# Autodesk Inventor assembly: 0304_練習
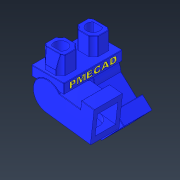
[picture p0: Inventor's stored thumbnail of the model, 180x180]
Saved by Autodesk Inventor 2022 (Build 260153000, 153)
## iProperties
Created: 2022-03-04
Part Number: 0304_練習
Document SubType Name: Assembly
Designer: user
Author: user
## Documents named in this file (4)
- D:\pomelo\大一\下學期\機械設計製圖\PME1017_110033226\0304_練習.iam
- D:\pomelo\大一\下學期\機械設計製圖\教材_LEGOmini_2022_20220218\X02598_LEGOmini_RightLeg_B.ipt
- D:\pomelo\大一\下學期\機械設計製圖\教材_LEGOmini_2022_20220218\X02598_LEGOmini_Waist_B.ipt
- D:\pomelo\大一\下學期\機械設計製圖\教材_LEGOmini_2022_20220218\X02598_LEGOmini_LeftLeg_B.ipt
## Components (3 placed, 3 different names)
1. X02598_LEGOmini_Waist_B:1 — 貼合:1, 貼合:2, 貼合:3, 貼合:4
2. X02598_LEGOmini_RightLeg_B:2 — 貼合:1, 貼合:2
3. X02598_LEGOmini_LeftLeg_B:1 — 貼合:3, 貼合:4
## Relationships (4: Mate 4)
- 貼合:1 [Mate]: X02598_LEGOmini_Waist_B:1 ↔ X02598_LEGOmini_RightLeg_B:2
- 貼合:2 [Mate]: X02598_LEGOmini_Waist_B:1 ↔ X02598_LEGOmini_RightLeg_B:2
- 貼合:3 [Mate]: X02598_LEGOmini_Waist_B:1 ↔ X02598_LEGOmini_LeftLeg_B:1
- 貼合:4 [Mate]: X02598_LEGOmini_Waist_B:1 ↔ X02598_LEGOmini_LeftLeg_B:1
